# Autodesk Inventor assembly: Completed Klaw Mechanism (Fully Assembled)
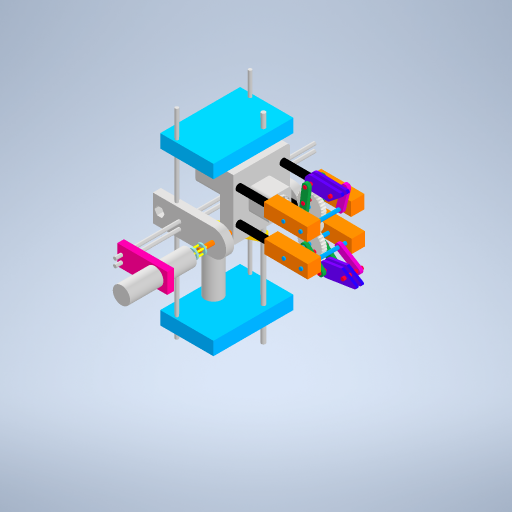
[picture p0: Inventor's stored thumbnail of the model, 512x512]
Saved by Autodesk Inventor 2023.1 (Build 271208000, 208)
## iProperties
Created: 2022-11-06
Part Number: Completed Klaw Mechanism (Fully Assembled)
Document SubType Name: Assembly
Designer: shubh
Author: shubh
## Documents named in this file (26)
- C:\Users\shubh\OneDrive\Desktop\Completed Klaw Mechanism\Completed Klaw Mechanism (Fully Assembled).iam
- C:\Users\shubh\OneDrive\Desktop\Completed Klaw Mechanism\Worm Gear1.ipt
- C:\Users\shubh\OneDrive\Desktop\Completed Klaw Mechanism\Worm1.ipt
- C:\Users\shubh\OneDrive\Desktop\Completed Klaw Mechanism\Gear to Finger Connect.ipt
- C:\Users\shubh\OneDrive\Desktop\Completed Klaw Mechanism\Finger.ipt
- C:\Users\shubh\OneDrive\Desktop\Completed Klaw Mechanism\shafts.ipt
- C:\Users\shubh\OneDrive\Desktop\Completed Klaw Mechanism\0.25_in_shaft.ipt
- C:\Users\shubh\OneDrive\Desktop\Completed Klaw Mechanism\Base.ipt
- C:\Users\shubh\OneDrive\Desktop\Completed Klaw Mechanism\Base to Finger Connect.ipt
- C:\Users\shubh\OneDrive\Desktop\Completed Klaw Mechanism\0.25 in long shaft.ipt
- C:\Users\shubh\OneDrive\Desktop\Completed Klaw Mechanism\Contracting Finger Motion Motot Mount.ipt
- C:\Users\shubh\OneDrive\Desktop\Completed Klaw Mechanism\Contracting Finger Motion Ring (shaft to motor).ipt
- C:\Users\shubh\OneDrive\Desktop\Completed Klaw Mechanism\Contracting Finger Motion Ring (motor to shaft).ipt
- C:\Users\shubh\OneDrive\Desktop\Completed Klaw Mechanism\Flip up and down motion motor mount.ipt
- C:\Users\shubh\OneDrive\Desktop\Completed Klaw Mechanism\Planetary Motor.ipt
- C:\Users\shubh\OneDrive\Desktop\Completed Klaw Mechanism\Flip up and down (motor to shaft ring).ipt
- C:\Users\shubh\OneDrive\Desktop\Completed Klaw Mechanism\0.313 in (6 in long) shaft.ipt
- C:\Users\shubh\OneDrive\Desktop\Completed Klaw Mechanism\Flip up and down (shaft to motor ring).ipt
- C:\Users\shubh\OneDrive\Desktop\Completed Klaw Mechanism\Top Plate for Side to Side motion.ipt
- C:\Users\shubh\OneDrive\Desktop\Completed Klaw Mechanism\Bottom Plate For Side to Side Motion.ipt
- C:\Users\shubh\OneDrive\Desktop\Completed Klaw Mechanism\Motor to Shaft Connection for Side to Side motion.ipt
- C:\Users\shubh\OneDrive\Desktop\Completed Klaw Mechanism\0.313 in shaft (15 in).ipt
- C:\Users\shubh\OneDrive\Desktop\Completed Klaw Mechanism\0.25 in shaft (15 in).ipt
- C:\Users\shubh\OneDrive\Desktop\Completed Klaw Mechanism\0.125 in shaft (1 in).ipt
- C:\Users\shubh\OneDrive\Desktop\Completed Klaw Mechanism\Real Yellow Jacket.ipt
- C:\Users\shubh\OneDrive\Desktop\Updated Files\new plates for arm.ipt
## Components (56 placed, 25 different names)
1. Worm Gear:1 — Flush:1, Mate:1, Rotation:1, Angle:1, Mate:3, Mate:4, Mate:5, Mate:6, Mate:7, Mate:8, Tangent:3, Flush:10
2. Worm:1 — Mate:2, Flush:2, Rotation:1, Insert:13, Tangent:3, Rotation:2, Tangent:4
3. Gear to Finger Connect:1 — Mate:3, Mate:4, Mate:5, Mate:14, Flush:5, Mate:15, Flush:7, Flush:9, Mate:34, Mate:81
4. Gear to Finger Connect:2 — Mate:6, Mate:7, Mate:8, Flush:6, Flush:8
5. shafts:1 — Insert:13, Mate:91, Flush:19
6. 0.25_in_shaft:2 — Mate:14, Flush:5, Flush:6
7. 0.25_in_shaft:3 — Mate:15, Flush:7, Flush:8, Mate:25, Mate:26
8. Base to Finger Connect:1 — Angle:3, Mate:24, Mate:29, Mate:61, Mate:62, Mate:90
9. Finger:3 — Mate:24, Flush:9, Mate:25, Mate:27, Mate:28, Mate:30, Mate:61
10. Finger:4 — Mate:26, Mate:27, Mate:28, Mate:31
11. 0.25_in_shaft:4 — Mate:29, Mate:30, Mate:31
12. 0.25 in long shaft:1 — Mate:34, Mate:59, Mate:76, Flush:14
13. Worm Gear:2 — Flush:10, Rotation:2, Tangent:4, Mate:63, Mate:64, Mate:65, Mate:66, Mate:67, Mate:68, Mate:74
14. Base:1 — Mate:59, Mate:62, Flush:12
15. Gear to Finger Connect:3 — Mate:63, Mate:64, Mate:67, Mate:69, Mate:70, Flush:11, Mate:79, Mate:88, Flush:17, Mate:89, Flush:18
16. Gear to Finger Connect:4 — Mate:65, Mate:66, Mate:68
17. Finger:5 — Mate:69, Mate:71, Mate:72, Flush:11, Mate:86, Mate:87
18. Finger:6 — Mate:70, Mate:71, Mate:72, Mate:73
19. Base to Finger Connect:2 — Mate:73, Mate:75, Mate:80
20. Base:2 — Mate:74, Flush:12, Mate:75
21. Base:3 — Mate:76, Mate:81, Flush:13, Mate:83, Mate:84
22. Base:4 — Mate:79, Mate:80, Flush:13, Mate:82, Mate:85, Flush:15
23. 0.25 in long shaft:2 — Mate:82, Flush:16
24. 0.25 in long shaft:3 — Mate:83, Mate:84, Flush:14, Mate:90
25. 0.25 in long shaft:4 — Mate:85, Flush:15, Flush:16
26. 0.25_in_shaft:5 — Mate:86, Mate:87
27. 0.25_in_shaft:6 — Mate:88, Flush:17
28. 0.25_in_shaft:7 — Mate:89, Flush:18
29. Contracting Finger Motion Ring (shaft to motor):1 — Mate:91, Flush:19, Mate:94, Mate:95, Mate:96
30. Contracting Finger Motion Motot Mount:1 — Mate:97, Mate:111, Flush:38, Mate:153, Mate:168
31. Contracting Finger Motion Ring (motor to shaft):1 — Mate:94, Mate:95, Mate:96, Mate:140, Mate:141, Mate:142, Mate:143, Flush:34, Flush:35, Flush:36, Flush:37, Mate:145, Mate:146
32. Planetary Motor:1 — Mate:104, Flush:23, Mate:112, Mate:113
33. Flip up and down (motor to shaft ring):1 — Mate:104, Flush:23, Mate:109, Mate:110, Mate:114, Mate:133, Mate:135, Mate:137, Mate:138, Flush:30, Flush:31, Flush:32, Flush:33
34. 0.313 in (6 in long) shaft:1 — Mate:107, Mate:108, Mate:111, Mate:147, Mate:155
35. Flip up and down (shaft to motor ring):1 — Mate:107, Mate:108, Mate:109, Mate:110, Mate:114, Mate:132, Mate:134, Mate:136, Mate:139
36. Flip up and down motion motor mount:1 — Mate:112, Mate:113, Mate:130, Mate:131, Mate:176, Flush:43, Flush:44, Angle:4
37. Planetary Motor:2 — Mate:171, Flush:41, Mate:172, Flush:42
38. 0.313 in shaft (15 in):1 — Mate:152, Mate:153, Mate:160, Mate:169, Mate:170, Mate:173
39. 0.25 in shaft (15 in):1 — Mate:149, Mate:161, Mate:174
40. 0.25 in shaft (15 in):2 — Mate:154, Mate:162
41. 0.25 in shaft (15 in):3 — Mate:130, Mate:176, Flush:43
42. 0.25 in shaft (15 in):4 — Mate:131, Flush:44
43. 0.125 in shaft (1 in):1 — Mate:136, Mate:137, Flush:32
44. 0.125 in shaft (1 in):2 — Mate:132, Mate:133, Flush:30
45. 0.125 in shaft (1 in):3 — Mate:134, Mate:135, Flush:31
46. 0.125 in shaft (1 in):4 — Mate:138, Mate:139, Flush:33
47. 0.125 in shaft (1 in):5 — Mate:141, Flush:37
48. 0.125 in shaft (1 in):6 — Mate:142, Flush:36
49. 0.125 in shaft (1 in):7 — Mate:143, Flush:35
50. 0.125 in shaft (1 in):8 — Mate:140, Flush:34
51. Real Yellow Jacket:1 — Mate:145, Flush:38, Mate:146, Mate:168
52. new plates for arm:1 — Mate:147, Mate:149, Angle:4
53. new plates for arm:2 — Mate:154, Mate:155
54. Bottom Plate For Side to Side Motion:1 — Mate:152, Mate:170, Mate:171, Flush:41, Mate:174, Mate:175
55. Top Plate for Side to Side motion:1 — Mate:160, Mate:161, Mate:162, Mate:169, Mate:175
56. Motor to Shaft Connection for Side to Side motion:1 — Mate:172, Mate:173, Flush:42
## Relationships (135: Mate 96, Flush 31, Angle 3, RelateRotation 2, Tangent 2, Insert 1)
- Flush:1: Worm Gear:1
- Mate:1: Worm Gear:1
- Mate:2: Worm:1
- Flush:2: Worm:1
- Rotation:1 [RelateRotation] (3 ul): Worm Gear:1 ↔ Worm:1
- Angle:1 (180 deg): Worm Gear:1
- Mate:3: Worm Gear:1 ↔ Gear to Finger Connect:1
- Mate:4: Worm Gear:1 ↔ Gear to Finger Connect:1
- Mate:5 (6.35 mm): Worm Gear:1 ↔ Gear to Finger Connect:1
- Mate:6: Worm Gear:1 ↔ Gear to Finger Connect:2
- Mate:7: Worm Gear:1 ↔ Gear to Finger Connect:2
- Mate:8 (6.35 mm): Worm Gear:1 ↔ Gear to Finger Connect:2
- Insert:13: Worm:1 ↔ shafts:1
- Mate:14: Gear to Finger Connect:1 ↔ 0.25_in_shaft:2
- Flush:5 (1.5748 mm): Gear to Finger Connect:1 ↔ 0.25_in_shaft:2
- Flush:6 (-1.5748 mm): Gear to Finger Connect:2 ↔ 0.25_in_shaft:2
- Mate:15: Gear to Finger Connect:1 ↔ 0.25_in_shaft:3
- Flush:7 (-1.5748 mm): Gear to Finger Connect:1 ↔ 0.25_in_shaft:3
- Flush:8 (-1.5748 mm): Gear to Finger Connect:2 ↔ 0.25_in_shaft:3
- Angle:3 (90 deg): Base to Finger Connect:1
- Mate:24: Base to Finger Connect:1 ↔ Finger:3
- Flush:9 (-20.32 mm): Gear to Finger Connect:1 ↔ Finger:3
- Mate:25: 0.25_in_shaft:3 ↔ Finger:3
- Mate:26: 0.25_in_shaft:3 ↔ Finger:4
- Mate:27: Finger:3 ↔ Finger:4
- Mate:28 (5.08 mm): Finger:3 ↔ Finger:4
- Mate:29: Base to Finger Connect:1 ↔ 0.25_in_shaft:4
- Mate:30: Finger:3 ↔ 0.25_in_shaft:4
- Mate:31 (3.81 mm): Finger:4 ↔ 0.25_in_shaft:4
- Mate:34: Gear to Finger Connect:1 ↔ 0.25 in long shaft:1
- Tangent:3: Worm Gear:1 ↔ Worm:1
- Flush:10: Worm Gear:1 ↔ Worm Gear:2
- Rotation:2 [RelateRotation] (3 ul): Worm:1 ↔ Worm Gear:2
- Tangent:4: Worm:1 ↔ Worm Gear:2
- Mate:59: 0.25 in long shaft:1 ↔ Base:1
- Mate:61 (10.16 mm): Base to Finger Connect:1 ↔ Finger:3
- Mate:62 (5.08 mm): Base to Finger Connect:1 ↔ Base:1
- Mate:63: Worm Gear:2 ↔ Gear to Finger Connect:3
- Mate:64: Worm Gear:2 ↔ Gear to Finger Connect:3
- Mate:65: Worm Gear:2 ↔ Gear to Finger Connect:4
- Mate:66: Worm Gear:2 ↔ Gear to Finger Connect:4
- Mate:67 (5.08 mm): Worm Gear:2 ↔ Gear to Finger Connect:3
- Mate:68 (5.08 mm): Worm Gear:2 ↔ Gear to Finger Connect:4
- Mate:69: Gear to Finger Connect:3 ↔ Finger:5
- Mate:70: Gear to Finger Connect:3 ↔ Finger:6
- Mate:71 (5.08 mm): Finger:5 ↔ Finger:6
- Mate:72: Finger:5 ↔ Finger:6
- Flush:11 (-8.89 mm): Gear to Finger Connect:3 ↔ Finger:5
- Mate:73: Finger:6 ↔ Base to Finger Connect:2
- Mate:74: Worm Gear:2 ↔ Base:2
- Flush:12: Base:1 ↔ Base:2
- Mate:75: Base to Finger Connect:2 ↔ Base:2
- Mate:76: 0.25 in long shaft:1 ↔ Base:3
- Mate:79: Gear to Finger Connect:3 ↔ Base:4
- Mate:80: Base to Finger Connect:2 ↔ Base:4
- Mate:81 (10.16 mm): Gear to Finger Connect:1 ↔ Base:3
- Flush:13: Base:3 ↔ Base:4
- Mate:82: Base:4 ↔ 0.25 in long shaft:2
- Mate:83: Base:3 ↔ 0.25 in long shaft:3
- Mate:84 (2.54 mm): Base:3 ↔ 0.25 in long shaft:3
- Flush:14 (-0.5842 mm): 0.25 in long shaft:1 ↔ 0.25 in long shaft:3
- Mate:85: Base:4 ↔ 0.25 in long shaft:4
- Flush:15 (2.54 mm): Base:4 ↔ 0.25 in long shaft:4
- Flush:16 (0.254 mm): 0.25 in long shaft:2 ↔ 0.25 in long shaft:4
- Mate:86: Finger:5 ↔ 0.25_in_shaft:5
- Mate:87 (5.08 mm): Finger:5 ↔ 0.25_in_shaft:5
- Mate:88: Gear to Finger Connect:3 ↔ 0.25_in_shaft:6
- Flush:17 (-2.54 mm): Gear to Finger Connect:3 ↔ 0.25_in_shaft:6
- Mate:89: Gear to Finger Connect:3 ↔ 0.25_in_shaft:7
- Flush:18 (-2.54 mm): Gear to Finger Connect:3 ↔ 0.25_in_shaft:7
- Mate:90: Base to Finger Connect:1 ↔ 0.25 in long shaft:3
- Mate:91: shafts:1 ↔ Contracting Finger Motion Ring (shaft to motor):1
- Flush:19 (-1.27 mm): shafts:1 ↔ Contracting Finger Motion Ring (shaft to motor):1
- Mate:94: Contracting Finger Motion Ring (shaft to motor):1 ↔ Contracting Finger Motion Ring (motor to shaft):1
- Mate:95: Contracting Finger Motion Ring (shaft to motor):1 ↔ Contracting Finger Motion Ring (motor to shaft):1
- Mate:96 (12.7 mm): Contracting Finger Motion Ring (shaft to motor):1 ↔ Contracting Finger Motion Ring (motor to shaft):1
- Mate:97: Contracting Finger Motion Motot Mount:1
- Mate:104: Planetary Motor:1 ↔ Flip up and down (motor to shaft ring):1
- Flush:23 (-4.445 mm): Planetary Motor:1 ↔ Flip up and down (motor to shaft ring):1
- Mate:107: 0.313 in (6 in long) shaft:1 ↔ Flip up and down (shaft to motor ring):1
- Mate:108 (-6.35 mm): 0.313 in (6 in long) shaft:1 ↔ Flip up and down (shaft to motor ring):1
- Mate:109: Flip up and down (motor to shaft ring):1 ↔ Flip up and down (shaft to motor ring):1
- Mate:110: Flip up and down (motor to shaft ring):1 ↔ Flip up and down (shaft to motor ring):1
- Mate:111: Contracting Finger Motion Motot Mount:1 ↔ 0.313 in (6 in long) shaft:1
- Mate:112: Planetary Motor:1 ↔ Flip up and down motion motor mount:1
- Mate:113: Planetary Motor:1 ↔ Flip up and down motion motor mount:1
- Mate:114 (12.7 mm): Flip up and down (motor to shaft ring):1 ↔ Flip up and down (shaft to motor ring):1
- Mate:130: Flip up and down motion motor mount:1 ↔ 0.25 in shaft (15 in):3
- Mate:131: Flip up and down motion motor mount:1 ↔ 0.25 in shaft (15 in):4
- Mate:132: Flip up and down (shaft to motor ring):1 ↔ 0.125 in shaft (1 in):2
- Mate:133: Flip up and down (motor to shaft ring):1 ↔ 0.125 in shaft (1 in):2
- Mate:134: Flip up and down (shaft to motor ring):1 ↔ 0.125 in shaft (1 in):3
- Mate:135: Flip up and down (motor to shaft ring):1 ↔ 0.125 in shaft (1 in):3
- Mate:136: Flip up and down (shaft to motor ring):1 ↔ 0.125 in shaft (1 in):1
- Mate:137: Flip up and down (motor to shaft ring):1 ↔ 0.125 in shaft (1 in):1
- Mate:138: Flip up and down (motor to shaft ring):1 ↔ 0.125 in shaft (1 in):4
- Mate:139: Flip up and down (shaft to motor ring):1 ↔ 0.125 in shaft (1 in):4
- Flush:30 (-3.81 mm): Flip up and down (motor to shaft ring):1 ↔ 0.125 in shaft (1 in):2
- Flush:31 (-3.81 mm): Flip up and down (motor to shaft ring):1 ↔ 0.125 in shaft (1 in):3
- Flush:32 (-3.81 mm): Flip up and down (motor to shaft ring):1 ↔ 0.125 in shaft (1 in):1
- Flush:33 (-3.81 mm): Flip up and down (motor to shaft ring):1 ↔ 0.125 in shaft (1 in):4
- Mate:140: Contracting Finger Motion Ring (motor to shaft):1 ↔ 0.125 in shaft (1 in):8
- Mate:141: Contracting Finger Motion Ring (motor to shaft):1 ↔ 0.125 in shaft (1 in):5
- Mate:142: Contracting Finger Motion Ring (motor to shaft):1 ↔ 0.125 in shaft (1 in):6
- Mate:143: Contracting Finger Motion Ring (motor to shaft):1 ↔ 0.125 in shaft (1 in):7
- Flush:34 (-3.175 mm): Contracting Finger Motion Ring (motor to shaft):1 ↔ 0.125 in shaft (1 in):8
- Flush:35 (-3.175 mm): Contracting Finger Motion Ring (motor to shaft):1 ↔ 0.125 in shaft (1 in):7
- Flush:36 (-3.175 mm): Contracting Finger Motion Ring (motor to shaft):1 ↔ 0.125 in shaft (1 in):6
- Flush:37 (-3.175 mm): Contracting Finger Motion Ring (motor to shaft):1 ↔ 0.125 in shaft (1 in):5
- Mate:145: Contracting Finger Motion Ring (motor to shaft):1 ↔ Real Yellow Jacket:1
- Flush:38 (-3.81 mm): Contracting Finger Motion Motot Mount:1 ↔ Real Yellow Jacket:1
- Mate:146 (-6.35 mm): Contracting Finger Motion Ring (motor to shaft):1 ↔ Real Yellow Jacket:1
- Mate:147: 0.313 in (6 in long) shaft:1 ↔ new plates for arm:1
- Mate:149: 0.25 in shaft (15 in):1 ↔ new plates for arm:1
- Mate:152: 0.313 in shaft (15 in):1 ↔ Bottom Plate For Side to Side Motion:1
- Mate:153: Contracting Finger Motion Motot Mount:1 ↔ 0.313 in shaft (15 in):1
- Mate:154: 0.25 in shaft (15 in):2 ↔ new plates for arm:2
- Mate:155: 0.313 in (6 in long) shaft:1 ↔ new plates for arm:2
- Mate:160: 0.313 in shaft (15 in):1 ↔ Top Plate for Side to Side motion:1
- Mate:161: 0.25 in shaft (15 in):1 ↔ Top Plate for Side to Side motion:1
- Mate:162: 0.25 in shaft (15 in):2 ↔ Top Plate for Side to Side motion:1
- Mate:168: Contracting Finger Motion Motot Mount:1 ↔ Real Yellow Jacket:1
- Mate:169: 0.313 in shaft (15 in):1 ↔ Top Plate for Side to Side motion:1
- Mate:170: 0.313 in shaft (15 in):1 ↔ Bottom Plate For Side to Side Motion:1
- Mate:171: Planetary Motor:2 ↔ Bottom Plate For Side to Side Motion:1
- Flush:41 (-5.08 mm): Planetary Motor:2 ↔ Bottom Plate For Side to Side Motion:1
- Mate:172: Planetary Motor:2 ↔ Motor to Shaft Connection for Side to Side motion:1
- Mate:173 (0.3048 mm): 0.313 in shaft (15 in):1 ↔ Motor to Shaft Connection for Side to Side motion:1
- Flush:42 (2.54 mm): Planetary Motor:2 ↔ Motor to Shaft Connection for Side to Side motion:1
- Mate:174: 0.25 in shaft (15 in):1 ↔ Bottom Plate For Side to Side Motion:1
- Mate:175 (266.7 mm): Bottom Plate For Side to Side Motion:1 ↔ Top Plate for Side to Side motion:1
- Mate:176: Flip up and down motion motor mount:1 ↔ 0.25 in shaft (15 in):3
- Flush:43 (-12.7 mm): Flip up and down motion motor mount:1 ↔ 0.25 in shaft (15 in):3
- Flush:44 (-12.7 mm): Flip up and down motion motor mount:1 ↔ 0.25 in shaft (15 in):4
- Angle:4 (180 deg): Flip up and down motion motor mount:1 ↔ new plates for arm:1
